# Autodesk Inventor assembly: V3Cata
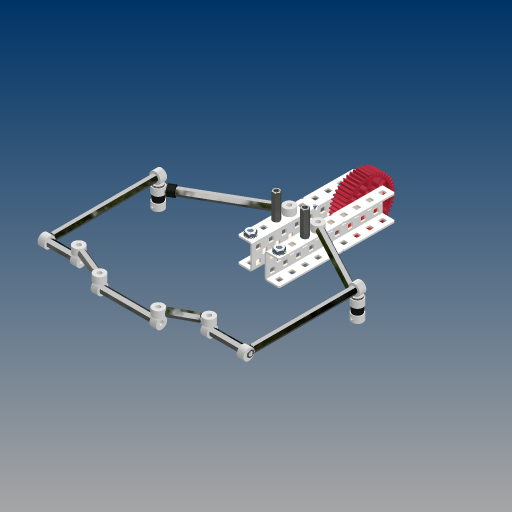
[picture p0: Inventor's stored thumbnail of the model, 512x512]
Saved by Autodesk Inventor 2023 (Build 270158000, 158)
## iProperties
Created: 2023-09-30
Part Number: V3Cata
Document SubType Name: Assembly
Designer: eddie
Author: eddie
## Documents named in this file (16)
- C:\Users\eddie\Documents\81208X-Over-Under-CAD\V3\V3Cata.iam
- C:\Users\eddie\Documents\81208X-Over-Under-CAD\VEX-CAD-Inventor-1.4.0\Structure\C Channel\Aluminum 1x2x1\Alu C 1x2x1x9.ipt
- C:\Users\eddie\Documents\81208X-Over-Under-CAD\VEX-CAD-Inventor-1.4.0\Structure\Hardware\Nut Keps.ipt
- C:\Users\eddie\Documents\81208X-Over-Under-CAD\VEX-CAD-Inventor-1.4.0\Structure\Standoff\Standoff 1.00.ipt
- C:\Users\eddie\Documents\81208X-Over-Under-CAD\VEX-CAD-Inventor-1.4.0\Structure\Standoff.ipt
- C:\Users\eddie\Documents\81208X-Over-Under-CAD\Custom-parts\Shaft Collar.ipt
- C:\Users\eddie\Documents\81208X-Over-Under-CAD\VEX-CAD-Inventor-1.4.0\Motion\Gears\HS Gear\HS 48T Gear, Square.iam
- C:\Users\eddie\Documents\81208X-Over-Under-CAD\VEX-CAD-Inventor-1.4.0\Motion\Gears\HS Gear.iam
- C:\Users\eddie\Documents\81208X-Over-Under-CAD\VEX-CAD-Inventor-1.4.0\Structure\Standoff\Standoff 3.00.ipt
- C:\Users\eddie\Documents\81208X-Over-Under-CAD\VEX-CAD-Inventor-1.4.0\Motion\Spacers\Spacer Nylon .375 OD\NSpacer .375 OD x .250.ipt
- C:\Users\eddie\Documents\81208X-Over-Under-CAD\VEX-CAD-Inventor-1.4.0\Motion\Spacers\Spacer Nylon .375 OD.ipt
- C:\Users\eddie\Documents\81208X-Over-Under-CAD\VEX-CAD-Inventor-1.4.0\Motion\Spacers\Washer Steel\SWasher .375 OD x .031250.ipt
- C:\Users\eddie\Documents\81208X-Over-Under-CAD\VEX-CAD-Inventor-1.4.0\Motion\Spacers\Washer Steel.ipt
- C:\Users\eddie\Documents\81208X-Over-Under-CAD\VEX-CAD-Inventor-1.4.0\Structure\Standoff\Standoff 4.00.ipt
- C:\Users\eddie\Documents\81208X-Over-Under-CAD\VEX-CAD-Inventor-1.4.0\Structure\Standoff\Standoff 2.00.ipt
- C:\Users\eddie\Documents\81208X-Over-Under-CAD\VEX-CAD-Inventor-1.4.0\Structure\Standoff\Standoff 1.50.ipt
## Components (45 placed, 11 different names)
1. Alu C 1x2x1x9:1 — Insert:1, Insert:9, Insert:13, Insert:15
2. Alu C 1x2x1x9:2 — Insert:2, Insert:10, Insert:12, Insert:14
3. Nut Keps:1 — Insert:1
4. Nut Keps:2 — Insert:2
5. Standoff 1.00:3 — Insert:10
6. Standoff 1.00:4 — Insert:9
7. Shaft Collar:1 — Insert:12, Insert:17
8. Shaft Collar:2 — Insert:13, Insert:16
9. HS 48T Gear, Square:1 [sub-assembly] — Insert:14, Insert:15
10. Standoff 3.00:5 — Insert:16, Insert:19
11. Standoff 3.00:6 — Insert:17, Insert:18
12. NSpacer .375 OD x .250:1 — Insert:18, Insert:21
13. NSpacer .375 OD x .250:2 — Insert:19, Insert:20
14. SWasher .375 OD x .031250:1 — Insert:21, Insert:22
15. SWasher .375 OD x .031250:2 — Insert:20, Insert:23
16. Shaft Collar:3 — Insert:23, Insert:24, Insert:32
17. Shaft Collar:4 — Insert:22, Insert:26, Insert:33
18. SWasher .375 OD x .031250:3 — Insert:26, Insert:27
19. SWasher .375 OD x .031250:4 — Insert:27, Insert:28
20. SWasher .375 OD x .031250:5 — Insert:25, Insert:29
21. SWasher .375 OD x .031250:6 — Insert:24, Insert:25
22. Shaft Collar:5 — Insert:28, Insert:30
23. Shaft Collar:6 — Insert:29, Insert:31
24. Standoff 4.00:7 — Insert:31, Insert:36
25. Standoff 4.00:8 — Insert:30, Insert:37
26. NSpacer .375 OD x .250:3 — Insert:32, Insert:34
27. NSpacer .375 OD x .250:4 — Insert:33, Insert:35
28. Shaft Collar:7 — Insert:34
29. Shaft Collar:8 — Insert:35
30. Shaft Collar:9 — Insert:37
31. Shaft Collar:10 — Insert:36, Insert:41
32. Standoff 1.00:11 — Insert:41, Insert:42
33. Standoff 1.00:12 — Insert:44, Insert:45
34. Shaft Collar:12 — Insert:42, Insert:43
35. Shaft Collar:13 — Insert:43, Insert:44
36. Shaft Collar:14 — Insert:45, Insert:46
37. Shaft Collar:15 — Insert:46, Insert:47
38. Standoff 2.00:15 — Insert:47, Insert:48
39. SWasher .375 OD x .031250:7 — Insert:48, Insert:49
40. Shaft Collar:16 — Insert:49, Insert:50
41. Shaft Collar:17 — Insert:50, Insert:51
42. Standoff 1.00:16 — Insert:51, Insert:52
43. Shaft Collar:18 — Insert:52, Insert:53
44. Shaft Collar:19 — Insert:53, Insert:54
45. Standoff 1.50:18 — Insert:54
## Relationships (44: Insert 44)
- Insert:1: Alu C 1x2x1x9:1 ↔ Nut Keps:1
- Insert:2: Alu C 1x2x1x9:2 ↔ Nut Keps:2
- Insert:9: Alu C 1x2x1x9:1 ↔ Standoff 1.00:4
- Insert:10: Alu C 1x2x1x9:2 ↔ Standoff 1.00:3
- Insert:12: Alu C 1x2x1x9:2 ↔ Shaft Collar:1
- Insert:13: Alu C 1x2x1x9:1 ↔ Shaft Collar:2
- Insert:14: Alu C 1x2x1x9:2 ↔ HS 48T Gear, Square:1
- Insert:15: Alu C 1x2x1x9:1 ↔ HS 48T Gear, Square:1
- Insert:16: Shaft Collar:2 ↔ Standoff 3.00:5
- Insert:17: Shaft Collar:1 ↔ Standoff 3.00:6
- Insert:18: Standoff 3.00:6 ↔ NSpacer .375 OD x .250:1
- Insert:19: Standoff 3.00:5 ↔ NSpacer .375 OD x .250:2
- Insert:20: NSpacer .375 OD x .250:2 ↔ SWasher .375 OD x .031250:2
- Insert:21: NSpacer .375 OD x .250:1 ↔ SWasher .375 OD x .031250:1
- Insert:22: SWasher .375 OD x .031250:1 ↔ Shaft Collar:4
- Insert:23: SWasher .375 OD x .031250:2 ↔ Shaft Collar:3
- Insert:24: Shaft Collar:3 ↔ SWasher .375 OD x .031250:6
- Insert:25: SWasher .375 OD x .031250:5 ↔ SWasher .375 OD x .031250:6
- Insert:26: Shaft Collar:4 ↔ SWasher .375 OD x .031250:3
- Insert:27: SWasher .375 OD x .031250:3 ↔ SWasher .375 OD x .031250:4
- Insert:28: SWasher .375 OD x .031250:4 ↔ Shaft Collar:5
- Insert:29: SWasher .375 OD x .031250:5 ↔ Shaft Collar:6
- Insert:30: Shaft Collar:5 ↔ Standoff 4.00:8
- Insert:31: Shaft Collar:6 ↔ Standoff 4.00:7
- Insert:32: Shaft Collar:3 ↔ NSpacer .375 OD x .250:3
- Insert:33: Shaft Collar:4 ↔ NSpacer .375 OD x .250:4
- Insert:34: NSpacer .375 OD x .250:3 ↔ Shaft Collar:7
- Insert:35: NSpacer .375 OD x .250:4 ↔ Shaft Collar:8
- Insert:36: Standoff 4.00:7 ↔ Shaft Collar:10
- Insert:37: Standoff 4.00:8 ↔ Shaft Collar:9
- Insert:41: Shaft Collar:10 ↔ Standoff 1.00:11
- Insert:42: Standoff 1.00:11 ↔ Shaft Collar:12
- Insert:43: Shaft Collar:12 ↔ Shaft Collar:13
- Insert:44: Standoff 1.00:12 ↔ Shaft Collar:13
- Insert:45: Standoff 1.00:12 ↔ Shaft Collar:14
- Insert:46: Shaft Collar:14 ↔ Shaft Collar:15
- Insert:47: Shaft Collar:15 ↔ Standoff 2.00:15
- Insert:48: Standoff 2.00:15 ↔ SWasher .375 OD x .031250:7
- Insert:49: SWasher .375 OD x .031250:7 ↔ Shaft Collar:16
- Insert:50: Shaft Collar:16 ↔ Shaft Collar:17
- Insert:51: Shaft Collar:17 ↔ Standoff 1.00:16
- Insert:52: Standoff 1.00:16 ↔ Shaft Collar:18
- Insert:53: Shaft Collar:18 ↔ Shaft Collar:19
- Insert:54: Shaft Collar:19 ↔ Standoff 1.50:18
